# Autodesk Inventor assembly: Tail_reallign
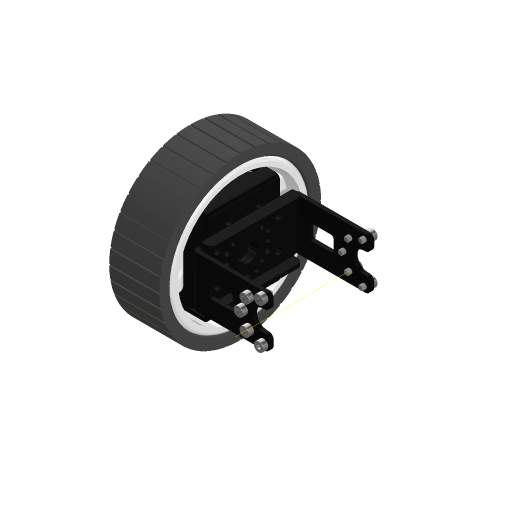
[picture p0: Inventor's stored thumbnail of the model, 512x512]
Saved by Autodesk Inventor 2024 (Build 280153000, 153)
## iProperties
Created: 2023-11-28
Part Number: Tail_reallign
Document SubType Name: Assembly
Designer: Bong
Mass: 50.9904 g
Surface Area: 322.99 cm^2
Volume: 49.2753 cm^3
Density: 1.03481 g/cm^3
Author: Bong
## Documents named in this file (7)
- C:\Users\Bong\project\snake_RL\matlab\meshes\Inventor_Reallign\tail\Tail_reallign.iam
- C:\Users\Bong\project\snake_RL\matlab\meshes\Inventor_Reallign\tail\xm430_hinge.ipt
- C:\Users\Bong\project\snake_RL\matlab\meshes\Inventor_Reallign\tail\xm430_tail_dummy.ipt
- C:\Users\Bong\project\snake_RL\matlab\meshes\Inventor_Reallign\tail\xm430_frame.ipt
- C:\Users\Bong\Documents\Inventor\Content Center Files\R2024\ko-KR\BS 4168(1)\BS 4168 - M2 x 3(1).ipt
- C:\Users\Bong\project\snake_RL\matlab\meshes\Inventor_Reallign\tail\solid_circular_frame_dummy.ipt
- C:\Users\Bong\project\snake_RL\matlab\meshes\Inventor_Reallign\tail\rubber.ipt
## Components (15 placed, 6 different names)
1. xm430_hinge:1 — 메이트:1, 메이트:3, 플러쉬:1, 강체:1, 강체:3, 강체:4, 강체:5, 강체:6, 강체:7, 강체:8, 강체:9, 강체:10, 강체:11, 강체:12, 강체:13
2. xm430_tail_dummy:1 — 강체:2
3. xm430_frame:1 — 강체:1, 강체:2
4. BS 4168 : 부품 1 6각 소켓 머리 캡 나사 - 미터 M2 x 3:1 — 강체:3
5. BS 4168 : 부품 1 6각 소켓 머리 캡 나사 - 미터 M2 x 3:2 — 강체:4
6. BS 4168 : 부품 1 6각 소켓 머리 캡 나사 - 미터 M2 x 3:3 — 강체:5
7. BS 4168 : 부품 1 6각 소켓 머리 캡 나사 - 미터 M2 x 3:4 — 강체:6
8. BS 4168 : 부품 1 6각 소켓 머리 캡 나사 - 미터 M2 x 3:5 — 강체:7
9. BS 4168 : 부품 1 6각 소켓 머리 캡 나사 - 미터 M2 x 3:6 — 강체:8
10. BS 4168 : 부품 1 6각 소켓 머리 캡 나사 - 미터 M2 x 3:7 — 강체:9
11. BS 4168 : 부품 1 6각 소켓 머리 캡 나사 - 미터 M2 x 3:8 — 강체:10
12. BS 4168 : 부품 1 6각 소켓 머리 캡 나사 - 미터 M2 x 3:9 — 강체:11
13. BS 4168 : 부품 1 6각 소켓 머리 캡 나사 - 미터 M2 x 3:10 — 강체:12
14. solid_circular_frame_dummy:1 — 강체:13, 강체:14
15. rubber:1 — 강체:14
## Relationships (18: WeldJoint 14, Mate 3, Flush 1)
- 메이트:1 [Mate]: xm430_hinge:1
- 메이트:2 [Mate]
- 메이트:3 [Mate]: xm430_hinge:1
- 플러쉬:1 [Flush]: xm430_hinge:1
- 강체:1 [WeldJoint]: xm430_hinge:1 ↔ xm430_frame:1
- 강체:2 [WeldJoint]: xm430_tail_dummy:1 ↔ xm430_frame:1
- 강체:3 [WeldJoint]: xm430_hinge:1 ↔ BS 4168 : 부품 1 6각 소켓 머리 캡 나사 - 미터 M2 x 3:1
- 강체:4 [WeldJoint]: xm430_hinge:1 ↔ BS 4168 : 부품 1 6각 소켓 머리 캡 나사 - 미터 M2 x 3:2
- 강체:5 [WeldJoint]: xm430_hinge:1 ↔ BS 4168 : 부품 1 6각 소켓 머리 캡 나사 - 미터 M2 x 3:3
- 강체:6 [WeldJoint]: xm430_hinge:1 ↔ BS 4168 : 부품 1 6각 소켓 머리 캡 나사 - 미터 M2 x 3:4
- 강체:7 [WeldJoint]: xm430_hinge:1 ↔ BS 4168 : 부품 1 6각 소켓 머리 캡 나사 - 미터 M2 x 3:5
- 강체:8 [WeldJoint]: xm430_hinge:1 ↔ BS 4168 : 부품 1 6각 소켓 머리 캡 나사 - 미터 M2 x 3:6
- 강체:9 [WeldJoint]: xm430_hinge:1 ↔ BS 4168 : 부품 1 6각 소켓 머리 캡 나사 - 미터 M2 x 3:7
- 강체:10 [WeldJoint]: xm430_hinge:1 ↔ BS 4168 : 부품 1 6각 소켓 머리 캡 나사 - 미터 M2 x 3:8
- 강체:11 [WeldJoint]: xm430_hinge:1 ↔ BS 4168 : 부품 1 6각 소켓 머리 캡 나사 - 미터 M2 x 3:9
- 강체:12 [WeldJoint]: xm430_hinge:1 ↔ BS 4168 : 부품 1 6각 소켓 머리 캡 나사 - 미터 M2 x 3:10
- 강체:13 [WeldJoint] (23 mm): xm430_hinge:1 ↔ solid_circular_frame_dummy:1
- 강체:14 [WeldJoint]: solid_circular_frame_dummy:1 ↔ rubber:1
